# Autodesk Inventor assembly: Montagem_Junta5
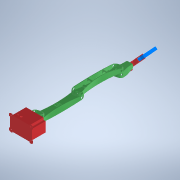
[picture p0: Inventor's stored thumbnail of the model, 180x180]
Saved by Autodesk Inventor 2021 (Build 250183000, 183)
## iProperties
Created: 2023-09-21
Part Number: Montagem_Junta5
Document SubType Name: Assembly
Designer: NOTEBOOK
Author: NOTEBOOK
## Documents named in this file (8)
- D:\LUAN\Semestre - Faculdade\PET\Projeto_Reuber_e_David\Testes_Garra\Montagem_Junta5.iam
- D:\LUAN\Semestre - Faculdade\PET\Projeto_Reuber_e_David\D2023\Braco Completo\BRAÇO ROBÓTICO - Base A1.ipt
- D:\LUAN\Semestre - Faculdade\PET\Projeto_Reuber_e_David\D2023\Braco Completo\BRAÇO ROBÓTICO - Base A2.ipt
- D:\LUAN\Semestre - Faculdade\PET\Projeto_Reuber_e_David\D2023\Braco Completo\BRAÇO ROBÓTICO - Base C2.ipt
- D:\LUAN\Semestre - Faculdade\PET\Projeto_Reuber_e_David\D2023\Braco Completo\BRAÇO ROBÓTICO - Braço B.ipt
- D:\LUAN\Semestre - Faculdade\PET\Projeto_Reuber_e_David\D2023\Braco Completo\BRAÇO ROBÓTICO - Braço A.ipt
- D:\LUAN\Semestre - Faculdade\PET\Projeto_Reuber_e_David\D2023\Braco Completo\BRAÇO ROBÓTICO - Braço C1.ipt
- D:\LUAN\Semestre - Faculdade\PET\Projeto_Reuber_e_David\Testes_Garra\garra_final.iam
## Components (7 placed, 7 different names)
1. BRAÇO ROBÓTICO - Base A1:1 — Rígida:1
2. BRAÇO ROBÓTICO - Base A2:1 — Rígida:1, Rotativa:1
3. BRAÇO ROBÓTICO - Base C2:1 — Rotativa:1, Rotativa:2
4. BRAÇO ROBÓTICO - Braço B:1 — Rotativa:2, Rotativa:3
5. BRAÇO ROBÓTICO - Braço A:1 — Rotativa:3, Rotativa:4
6. BRAÇO ROBÓTICO - Braço C1:1 — Rotativa:4, Inserir:1
7. garra_final:1 [sub-assembly] — Inserir:1
## Relationships (6: RevoluteJoint 4, WeldJoint 1, Insert 1)
- Rígida:1 [WeldJoint] (59.5 mm): BRAÇO ROBÓTICO - Base A1:1 ↔ BRAÇO ROBÓTICO - Base A2:1
- Rotativa:1 [RevoluteJoint]: BRAÇO ROBÓTICO - Base A2:1 ↔ BRAÇO ROBÓTICO - Base C2:1
- Rotativa:2 [RevoluteJoint]: BRAÇO ROBÓTICO - Base C2:1 ↔ BRAÇO ROBÓTICO - Braço B:1
- Rotativa:3 [RevoluteJoint]: BRAÇO ROBÓTICO - Braço B:1 ↔ BRAÇO ROBÓTICO - Braço A:1
- Rotativa:4 [RevoluteJoint]: BRAÇO ROBÓTICO - Braço A:1 ↔ BRAÇO ROBÓTICO - Braço C1:1
- Inserir:1: BRAÇO ROBÓTICO - Braço C1:1 ↔ garra_final:1
